# Autodesk Inventor assembly: Plstic Box Rear A Assembly with Battery Spacers
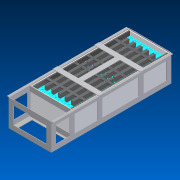
[picture p0: Inventor's stored thumbnail of the model, 180x180]
Saved by Autodesk Inventor 2012 (Build 160160000, 160)
## iProperties
Created: 2012-07-02
Part Number: Plstic Box Rear A Assembly with Battery Spacers
Document SubType Name: Assembly
Designer: Hemant
Author: Hemant
## Documents named in this file (4)
- C:\Users\Hemant\Documents\Battery Boxes\BB REAR A\Full Assembly.iam
- C:\Users\Hemant\Documents\Battery Boxes\BB REAR A\BB REAR B METAL ASSEMBLY\BB REAR B METAL Assembly.iam
- C:\Users\Hemant\Documents\Battery Boxes\BB REAR A\Plastic Box with Batteries and Spacer.iam
- C:\Users\Hemant\Documents\Battery Boxes\BB REAR A\Metal Lead\metal lead.iam
## Components (3 placed, 3 different names)
1. BB REAR B METAL Assembly:1 [sub-assembly] — Mate:1, Mate:2, Mate:3, Mate:4, Flush:1
2. Plastic Box with Batteries and Spacer:1 [sub-assembly] — Mate:1, Mate:2, Mate:3
3. metal lead:1 [sub-assembly] — Mate:4, Flush:1
## Relationships (5: Mate 4, Flush 1)
- Mate:1: BB REAR B METAL Assembly:1 ↔ Plastic Box with Batteries and Spacer:1
- Mate:2 (3.175 mm): BB REAR B METAL Assembly:1 ↔ Plastic Box with Batteries and Spacer:1
- Mate:3 (3.175 mm): BB REAR B METAL Assembly:1 ↔ Plastic Box with Batteries and Spacer:1
- Mate:4: BB REAR B METAL Assembly:1 ↔ metal lead:1
- Flush:1: BB REAR B METAL Assembly:1 ↔ metal lead:1
